# Autodesk Inventor assembly: reductor
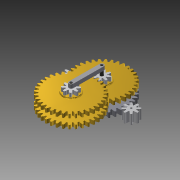
[picture p0: Inventor's stored thumbnail of the model, 180x180]
Saved by Autodesk Inventor 2014 SP1 (Build 180222100, 222)
## iProperties
Created: 2017-09-24
Part Number: reductor
Document SubType Name: Assembly
Designer: Vivi
Author: Vivi
## Documents named in this file (6)
- C:\Users\Vivi\Documents\Inventor\afinador falso\Imported Components\Sbdl\reductor.iam
- C:\Users\Vivi\Documents\Inventor\afinador falso\Imported Components\Sbdl\1streducction\Design Accelerator\Spur Gears1.iam
- C:\Users\Vivi\Documents\Inventor\afinador falso\Imported Components\Sbdl\engrane 1.iam
- C:\Users\Vivi\Documents\Inventor\afinador falso\Imported Components\Sbdl\1streducction\Design Accelerator\2ndreductor.ipt
- C:\Users\Vivi\Documents\Inventor\afinador falso\Imported Components\Sbdl\eje20.ipt
- C:\Users\Vivi\Documents\Inventor\afinador falso\Imported Components\Sbdl\un.ipt
## Components (9 placed, 5 different names)
1. Spur Gears:1 [sub-assembly] — Flush:1, Flush:2, Mate:1, Mate:6
2. engrane 1:1 [sub-assembly] — Flush:2
3. engrane 1:2 [sub-assembly] — Flush:1
4. Spur Gear1:1 — Mate:1, Mate:2, Mate:8
5. Spur Gear1:2 — Mate:2, Mate:3, Mate:5
6. Spur Gear1:3 — Mate:3, Mate:9
7. eje20:1 — Mate:5, Mate:6, Mate:7
8. un:1 — Mate:7, Mate:10
9. eje20:2 — Mate:8, Mate:9, Mate:10
## Relationships (11: Mate 9, Flush 2)
- Flush:1: Spur Gears:1 ↔ engrane 1:2
- Flush:2: Spur Gears:1 ↔ engrane 1:1
- Mate:1: Spur Gears:1 ↔ Spur Gear1:1
- Mate:2: Spur Gear1:1 ↔ Spur Gear1:2
- Mate:3: Spur Gear1:2 ↔ Spur Gear1:3
- Mate:5: Spur Gear1:2 ↔ eje20:1
- Mate:6: Spur Gears:1 ↔ eje20:1
- Mate:7: eje20:1 ↔ un:1
- Mate:8: Spur Gear1:1 ↔ eje20:2
- Mate:9: Spur Gear1:3 ↔ eje20:2
- Mate:10: un:1 ↔ eje20:2
